# Autodesk Inventor assembly: sliding block
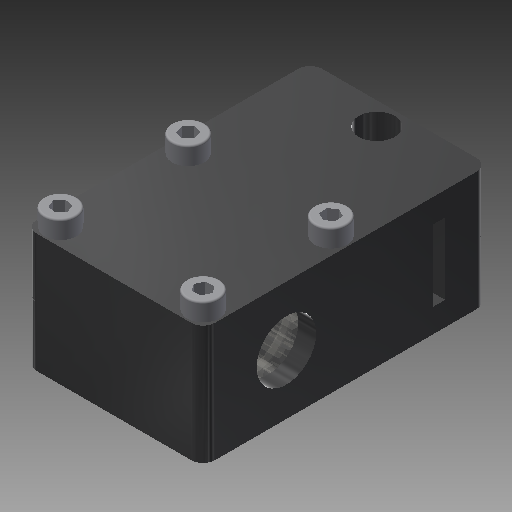
[picture p0: Inventor's stored thumbnail of the model, 512x512]
Saved by Autodesk Inventor 2017 (Build 210142000, 142)
## iProperties
Part Number: sliding block
Material: Generisch
Document SubType Name: Assembly
Designer: Till
Author: Till
## Documents named in this file (4)
- C:\Users\Till\Dropbox\DIY\CoreBot\sliding block.iam
- C:\Users\Till\Dropbox\DIY\CoreBot\Lagerblock XY.ipt
- C:\Users\Till\Dropbox\DIY\CoreBot\CAD Parts\IGUS RJ4JP.ipt
- C:\Users\Till\Dropbox\DIY\CoreBot\CAD Parts\item_0_0_616_29_6rrjpzm9kai2q6ysfss7799ws.ipt
## Components (7 placed, 3 different names)
1. Lagerblock XY:1 — Passend:1, Passend:2, Passend:3, Fluchtend:1, Fluchtend:2, Passend:4, Passend:5, Passend:6, Passend:7
2. IGUS RJ4JP:1 — Passend:1, Passend:2
3. Lagerblock XY:2 — Passend:3, Fluchtend:1, Fluchtend:2, Passend:10, Passend:11, Passend:9, Passend:8
4. item_0_0_616_29_6rrjpzm9kai2q6ysfss7799ws:1 — Passend:7, Passend:9
5. item_0_0_616_29_6rrjpzm9kai2q6ysfss7799ws:2 — Passend:6, Passend:10
6. item_0_0_616_29_6rrjpzm9kai2q6ysfss7799ws:3 — Passend:5, Passend:8
7. item_0_0_616_29_6rrjpzm9kai2q6ysfss7799ws:4 — Passend:4, Passend:11
## Relationships (13: Mate 11, Flush 2)
- Passend:1 [Mate]: Lagerblock XY:1 ↔ IGUS RJ4JP:1
- Passend:2 [Mate]: Lagerblock XY:1 ↔ IGUS RJ4JP:1
- Passend:3 [Mate]: Lagerblock XY:1 ↔ Lagerblock XY:2
- Fluchtend:1 [Flush]: Lagerblock XY:1 ↔ Lagerblock XY:2
- Fluchtend:2 [Flush]: Lagerblock XY:1 ↔ Lagerblock XY:2
- Passend:4 [Mate]: Lagerblock XY:1 ↔ item_0_0_616_29_6rrjpzm9kai2q6ysfss7799ws:4
- Passend:5 [Mate]: Lagerblock XY:1 ↔ item_0_0_616_29_6rrjpzm9kai2q6ysfss7799ws:3
- Passend:6 [Mate]: Lagerblock XY:1 ↔ item_0_0_616_29_6rrjpzm9kai2q6ysfss7799ws:2
- Passend:7 [Mate]: Lagerblock XY:1 ↔ item_0_0_616_29_6rrjpzm9kai2q6ysfss7799ws:1
- Passend:8 [Mate]: Lagerblock XY:2 ↔ item_0_0_616_29_6rrjpzm9kai2q6ysfss7799ws:3
- Passend:9 [Mate]: Lagerblock XY:2 ↔ item_0_0_616_29_6rrjpzm9kai2q6ysfss7799ws:1
- Passend:10 [Mate]: Lagerblock XY:2 ↔ item_0_0_616_29_6rrjpzm9kai2q6ysfss7799ws:2
- Passend:11 [Mate]: Lagerblock XY:2 ↔ item_0_0_616_29_6rrjpzm9kai2q6ysfss7799ws:4
